# Autodesk Inventor assembly: Drive Motor Assembly
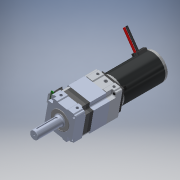
[picture p0: Inventor's stored thumbnail of the model, 180x180]
Saved by Autodesk Inventor 2019 (Build 230136000, 136)
## iProperties
Created: 2018-10-23
Part Number: Drive Motor Assembly
Document SubType Name: Assembly
Designer: Swapnil
Mass: 193.007 g
Surface Area: 930.591 cm^2
Volume: 193.007 cm^3
Density: 1 g/cm^3
Author: Swapnil
## Documents named in this file (16)
- C:\Users\Swapnil\Desktop\ImportantThings\Robotics\Vanderbilt Robotics\2018-2019\FrameAndDrive\DriveMotor\Drive Motor Assembly.iam
- C:\Users\Swapnil\Desktop\ImportantThings\Robotics\Vanderbilt Robotics\2018-2019\CAD\Bag Motor Assembly\217-3351 Rev2.ipt
- C:\Users\Swapnil\Desktop\ImportantThings\Robotics\Vanderbilt Robotics\2018-2019\CAD\Bag Motor Assembly\217-2822-003 Rev4.ipt
- C:\Users\Swapnil\Desktop\ImportantThings\Robotics\Vanderbilt Robotics\2018-2019\FrameAndDrive\DriveMotor\MotorScrews.ipt
- C:\Users\Swapnil\Desktop\ImportantThings\Robotics\Vanderbilt Robotics\2018-2019\FrameAndDrive\DriveMotor\MotorShaftGear.ipt
- C:\Users\Swapnil\Desktop\ImportantThings\Robotics\Vanderbilt Robotics\2018-2019\CAD\Bag Motor Assembly\217-2625-011 Rev1.ipt
- C:\Users\Swapnil\Desktop\ImportantThings\Robotics\Vanderbilt Robotics\2018-2019\CAD\Bag Motor Assembly\217-4649-007 Rev1_94105A824.ipt
- C:\Users\Swapnil\Desktop\ImportantThings\Robotics\Vanderbilt Robotics\2018-2019\FrameAndDrive\DriveMotor\FacePlateGearboxShortScrews.ipt
- C:\Users\Swapnil\Desktop\ImportantThings\Robotics\Vanderbilt Robotics\2018-2019\FrameAndDrive\DriveMotor\MotorMountSpacer.ipt
- C:\Users\Swapnil\Desktop\ImportantThings\Robotics\Vanderbilt Robotics\2018-2019\FrameAndDrive\DriveMotor\VersaPlanetary_10_1_Gear_Kit_217-2820.iam
- C:\Users\Swapnil\Desktop\ImportantThings\Robotics\Vanderbilt Robotics\2018-2019\FrameAndDrive\DriveMotor\RingGear.ipt
- C:\Users\Swapnil\Desktop\ImportantThings\Robotics\Vanderbilt Robotics\2018-2019\FrameAndDrive\DriveMotor\GearBoxOutputPlate.ipt
- C:\Users\Swapnil\Desktop\ImportantThings\Robotics\Vanderbilt Robotics\2018-2019\CAD\Bag Motor Assembly\VersaPlanetary_Integrated_Encoder_217-5046.iam
- C:\Users\Swapnil\Desktop\ImportantThings\Robotics\Vanderbilt Robotics\2018-2019\FrameAndDrive\DriveMotor\VersaPlanetary_1_2_with_1_8_Keyway_Output_Shaft_217-2895.ipt
- C:\Users\Swapnil\Desktop\ImportantThings\Robotics\Vanderbilt Robotics\2018-2019\FrameAndDrive\DriveMotor\OutputBearing.ipt
- C:\Users\Swapnil\Desktop\ImportantThings\Robotics\Vanderbilt Robotics\2018-2019\FrameAndDrive\DriveMotor\VersaPlanetary_10_1_Gear_Kit_217-2820.ipt
## Components (19 placed, 14 different names)
1. 217-3351 Rev2:1 — Mate:1, Mate:2, Mate:3, Mate:4, Mate:7, Mate:9, Mate:23
2. 217-2822-003 Rev4:1 — Mate:1, Mate:2, Mate:3, Mate:5, Mate:6, Mate:8, Mate:13, Mate:14, Mate:15, Mate:16, Mate:22, Flush:1
3. MotorScrews:1 — Mate:4, Mate:5
4. MotorScrews:2 — Mate:6, Mate:7
5. MotorShaftGear:1 — Mate:8, Mate:9, Mate:10, Mate:11, Mate:12, Mate:19
6. 217-2625-011 Rev1:1 — Mate:10, Mate:11
7. 217-4649-007 Rev1_94105A824:1 — Mate:12
8. FacePlateGearboxShortScrews:1 — Mate:13, Mate:14
9. FacePlateGearboxShortScrews:2 — Mate:15, Mate:16
10. MotorMountSpacer:1 — Mate:22, Mate:23, Flush:1, Mate:24, Mate:26
11. VersaPlanetary_10_1_Gear_Kit_217-2820:1 [sub-assembly] — Mate:19, Mate:25, Mate:42
12. RingGear:1 — Mate:24, Mate:25, Mate:26, Mate:27, Mate:29
13. RingGear:2 — Mate:27, Mate:29, Mate:43
14. VersaPlanetary_Integrated_Encoder_217-5046:1 [sub-assembly] — Mate:36, Mate:37, Mate:38, Mate:40, Mate:43
15. VersaPlanetary_1_2_with_1_8_Keyway_Output_Shaft_217-2895:1 — Mate:36, Mate:37, Mate:39, Mate:41
16. GearBoxOutputPlate:1 — Mate:38, Mate:39, Mate:40, Flush:2, Flush:3
17. OutputBearing:1 — Flush:2
18. OutputBearing:2 — Mate:41, Flush:3
19. VersaPlanetary_10_1_Gear_Kit_217-2820:2 — Mate:42
## Relationships (35: Mate 32, Flush 3)
- Mate:1: 217-3351 Rev2:1 ↔ 217-2822-003 Rev4:1
- Mate:2: 217-3351 Rev2:1 ↔ 217-2822-003 Rev4:1
- Mate:3: 217-3351 Rev2:1 ↔ 217-2822-003 Rev4:1
- Mate:4: 217-3351 Rev2:1 ↔ MotorScrews:1
- Mate:5: 217-2822-003 Rev4:1 ↔ MotorScrews:1
- Mate:6: 217-2822-003 Rev4:1 ↔ MotorScrews:2
- Mate:7: 217-3351 Rev2:1 ↔ MotorScrews:2
- Mate:8: 217-2822-003 Rev4:1 ↔ MotorShaftGear:1
- Mate:9: 217-3351 Rev2:1 ↔ MotorShaftGear:1
- Mate:10: MotorShaftGear:1 ↔ 217-2625-011 Rev1:1
- Mate:11: MotorShaftGear:1 ↔ 217-2625-011 Rev1:1
- Mate:12: MotorShaftGear:1 ↔ 217-4649-007 Rev1_94105A824:1
- Mate:13: 217-2822-003 Rev4:1 ↔ FacePlateGearboxShortScrews:1
- Mate:14: 217-2822-003 Rev4:1 ↔ FacePlateGearboxShortScrews:1
- Mate:15: 217-2822-003 Rev4:1 ↔ FacePlateGearboxShortScrews:2
- Mate:16: 217-2822-003 Rev4:1 ↔ FacePlateGearboxShortScrews:2
- Mate:19: MotorShaftGear:1 ↔ VersaPlanetary_10_1_Gear_Kit_217-2820:1
- Mate:22: 217-2822-003 Rev4:1 ↔ MotorMountSpacer:1
- Mate:23: 217-3351 Rev2:1 ↔ MotorMountSpacer:1
- Flush:1: 217-2822-003 Rev4:1 ↔ MotorMountSpacer:1
- Mate:24: MotorMountSpacer:1 ↔ RingGear:1
- Mate:25: VersaPlanetary_10_1_Gear_Kit_217-2820:1 ↔ RingGear:1
- Mate:26: MotorMountSpacer:1 ↔ RingGear:1
- Mate:27: RingGear:1 ↔ RingGear:2
- Mate:29: RingGear:1 ↔ RingGear:2
- Mate:36: VersaPlanetary_Integrated_Encoder_217-5046:1 ↔ VersaPlanetary_1_2_with_1_8_Keyway_Output_Shaft_217-2895:1
- Mate:37: VersaPlanetary_Integrated_Encoder_217-5046:1 ↔ VersaPlanetary_1_2_with_1_8_Keyway_Output_Shaft_217-2895:1
- Mate:38: VersaPlanetary_Integrated_Encoder_217-5046:1 ↔ GearBoxOutputPlate:1
- Mate:39: VersaPlanetary_1_2_with_1_8_Keyway_Output_Shaft_217-2895:1 ↔ GearBoxOutputPlate:1
- Mate:40: VersaPlanetary_Integrated_Encoder_217-5046:1 ↔ GearBoxOutputPlate:1
- Flush:2: GearBoxOutputPlate:1 ↔ OutputBearing:1
- Mate:41: VersaPlanetary_1_2_with_1_8_Keyway_Output_Shaft_217-2895:1 ↔ OutputBearing:2
- Flush:3: GearBoxOutputPlate:1 ↔ OutputBearing:2
- Mate:42: VersaPlanetary_10_1_Gear_Kit_217-2820:1 ↔ VersaPlanetary_10_1_Gear_Kit_217-2820:2
- Mate:43: RingGear:2 ↔ VersaPlanetary_Integrated_Encoder_217-5046:1
